# Autodesk Inventor assembly: Dribbler_Type2
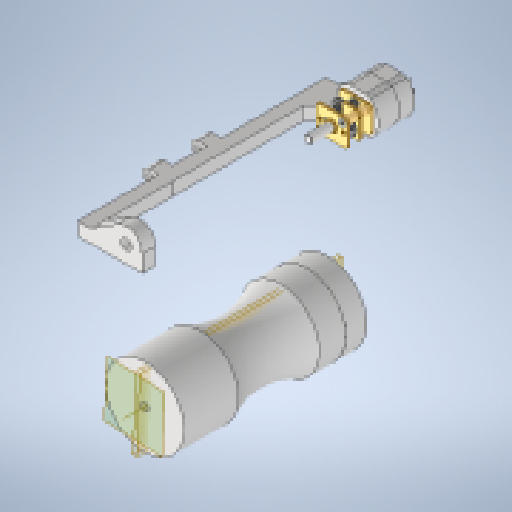
[picture p0: Inventor's stored thumbnail of the model, 512x512]
Saved by Autodesk Inventor 2025.1 (Build 291241000, 241)
## iProperties
Created: 2026-05-05
Part Number: Dribbler_Type2
Document SubType Name: Assembly
Designer: User
Author: User
## Documents named in this file (4)
- D:\One Drive\OneDrive - Politeknik Sultan Salahuddin Abdul Aziz Shah\Documents\Inventor\RobosotPSA\Dribbler_Type2.iam
- D:\One Drive\OneDrive - Politeknik Sultan Salahuddin Abdul Aziz Shah\Documents\Inventor\RobosotPSA\Drib_v2.ipt
- D:\One Drive\OneDrive - Politeknik Sultan Salahuddin Abdul Aziz Shah\Documents\Inventor\RobosotPSA\N20 Mini Micro Metall Gear Motor DC 3-6-12V v1\N20 Mini Micro Metall Gear Motor DC 3-6-12V v1\N20 Mini Micro Me.ipt
- D:\One Drive\OneDrive - Politeknik Sultan Salahuddin Abdul Aziz Shah\Documents\Inventor\RobosotPSA\Roller_Drib_v2.ipt
## Components (3 placed, 3 different names)
1. Drib_v2:1 — Mate:1, Mate:2
2. N20 Mini Micro Me:2
3. Roller_Drib_v2:1 — Mate:1, Mate:2
## Relationships (2: Mate 2)
- Mate:1: Drib_v2:1 ↔ Roller_Drib_v2:1
- Mate:2 (1.5 mm): Drib_v2:1 ↔ Roller_Drib_v2:1
